# Autodesk Inventor assembly: 200-10-ROCKER-BEARING-ASM-01
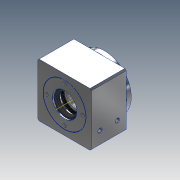
[picture p0: Inventor's stored thumbnail of the model, 180x180]
Saved by Autodesk Inventor 2018.1 (Build 221171000, 171)
## iProperties
Created: 2017-10-26
Part Number: 200-10-ROCKER-BEARING-ASM-01
Document SubType Name: Assembly
Designer: marti
Mass: 1761.19 g
Surface Area: 1330.32 cm^2
Volume: 535.142 cm^3
Density: 3.29106 g/cm^3
Author: marti
## Documents named in this file (8)
- C:\Users\feesmrt\Documents\NRBDL\Inventor-NRBDL\02-Rocker-Bogie-Robot\200-ROCKER-BOGIE\200-10-ROCKER-BEARING-ASM-01.iam
- C:\Users\feesmrt\Documents\NRBDL\Inventor-NRBDL\02-Rocker-Bogie-Robot\200-ROCKER-BOGIE\200-10-ROCKER-BEARING-01.ipt
- C:\Users\feesmrt\Documents\NRBDL\Inventor-NRBDL\02-Rocker-Bogie-Robot\900-COMPONENTS\900-20-BEARINGS\900-20-BEARINGS-3306-2RS-TN.ipt
- C:\Users\feesmrt\Documents\NRBDL\Inventor-NRBDL\02-Rocker-Bogie-Robot\200-ROCKER-BOGIE\200-10-ROCKER-BEARING-02.ipt
- C:\Users\feesmrt\Documents\NRBDL\Inventor-NRBDL\02-Rocker-Bogie-Robot\900-COMPONENTS\900-30-SEALS\900-30-SEALS-DIN-3760-AS38x55x8-NBR.ipt
- C:\Users\feesmrt\Documents\NRBDL\Inventor-NRBDL\02-Rocker-Bogie-Robot\200-ROCKER-BOGIE\200-10-ROCKER-BEARING-03.ipt
- C:\Users\feesmrt\Documents\NRBDL\Inventor-NRBDL\02-Rocker-Bogie-Robot\900-COMPONENTS\900-40-SCREWS\900-40-SCREWS-ISO4762_M6x12.ipt
- C:\Users\feesmrt\Documents\NRBDL\Inventor-NRBDL\02-Rocker-Bogie-Robot\900-COMPONENTS\900-40-SCREWS\900-40-SCREWS-ISO10642_M3x8.ipt
## Components (15 placed, 7 different names)
1. 200-10-ROCKER-BEARING-01:1 — Passend:1, Passend:2, Passend:3, Passend:6, Passend:7, Passend:8, Passend:9, Passend:10, Passend:11, Passend:14, Passend:15
2. 900-20-BEARINGS-3306-2RS-TN:1 — Passend:1, Passend:2, Passend:3, Passend:4
3. 200-10-ROCKER-BEARING-02:1 — Passend:4, Passend:6, Passend:15, Passend:16, Passend:17
4. 900-30-SEALS-DIN-3760-AS38x55x8-NBR:1 — Passend:7, Passend:8
5. 200-10-ROCKER-BEARING-03:1 — Passend:9, Passend:10, Passend:11, Fluchtend:1
6. 900-40-SCREWS-ISO10642_M3x8:1 — Fluchtend:1, Passend:14
7. 900-40-SCREWS-ISO10642_M3x8:2
8. 900-40-SCREWS-ISO10642_M3x8:3
9. 900-40-SCREWS-ISO10642_M3x8:4
10. 900-40-SCREWS-ISO4762_M6x12:1 — Passend:16, Passend:17
11. 900-40-SCREWS-ISO4762_M6x12:2
12. 900-40-SCREWS-ISO4762_M6x12:3
13. 900-40-SCREWS-ISO4762_M6x12:4
14. 900-40-SCREWS-ISO4762_M6x12:5
15. 900-40-SCREWS-ISO4762_M6x12:6
## Component patterns: ISO10642_M3x8 (4 elements), ISO4762_M6x12 (6 elements)
## Relationships (15: Mate 14, Flush 1)
- Passend:1 [Mate]: 200-10-ROCKER-BEARING-01:1 ↔ 900-20-BEARINGS-3306-2RS-TN:1
- Passend:2 [Mate]: 200-10-ROCKER-BEARING-01:1 ↔ 900-20-BEARINGS-3306-2RS-TN:1
- Passend:3 [Mate]: 200-10-ROCKER-BEARING-01:1 ↔ 900-20-BEARINGS-3306-2RS-TN:1
- Passend:4 [Mate]: 900-20-BEARINGS-3306-2RS-TN:1 ↔ 200-10-ROCKER-BEARING-02:1
- Passend:6 [Mate]: 200-10-ROCKER-BEARING-01:1 ↔ 200-10-ROCKER-BEARING-02:1
- Passend:7 [Mate]: 200-10-ROCKER-BEARING-01:1 ↔ 900-30-SEALS-DIN-3760-AS38x55x8-NBR:1
- Passend:8 [Mate]: 200-10-ROCKER-BEARING-01:1 ↔ 900-30-SEALS-DIN-3760-AS38x55x8-NBR:1
- Passend:9 [Mate]: 200-10-ROCKER-BEARING-01:1 ↔ 200-10-ROCKER-BEARING-03:1
- Passend:10 [Mate]: 200-10-ROCKER-BEARING-01:1 ↔ 200-10-ROCKER-BEARING-03:1
- Passend:11 [Mate]: 200-10-ROCKER-BEARING-01:1 ↔ 200-10-ROCKER-BEARING-03:1
- Fluchtend:1 [Flush]: 200-10-ROCKER-BEARING-03:1 ↔ 900-40-SCREWS-ISO10642_M3x8:1
- Passend:14 [Mate]: 200-10-ROCKER-BEARING-01:1 ↔ 900-40-SCREWS-ISO10642_M3x8:1
- Passend:15 [Mate]: 200-10-ROCKER-BEARING-01:1 ↔ 200-10-ROCKER-BEARING-02:1
- Passend:16 [Mate]: 200-10-ROCKER-BEARING-02:1 ↔ 900-40-SCREWS-ISO4762_M6x12:1
- Passend:17 [Mate]: 200-10-ROCKER-BEARING-02:1 ↔ 900-40-SCREWS-ISO4762_M6x12:1
